# Autodesk Inventor assembly: M2-M-前足
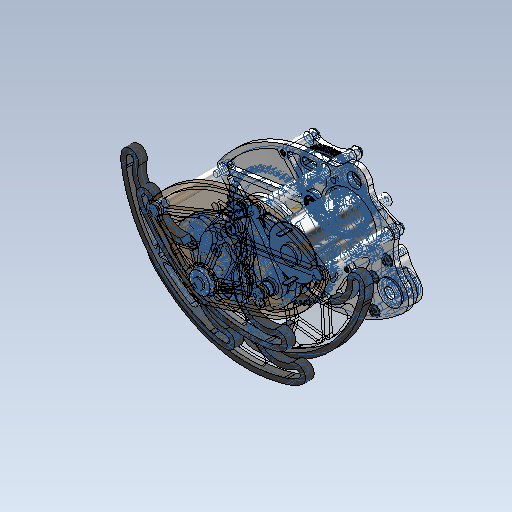
[picture p0: Inventor's stored thumbnail of the model, 512x512]
Saved by Autodesk Inventor 2020 (Build 240168000, 168)
## iProperties
Created: 2021-02-23
Part Number: M2-M-前足
Document SubType Name: Assembly
Designer: AA19065
Mass: 271.583 g
Surface Area: 1202.67 cm^2
Volume: 103.505 cm^3
Density: 2.62385 g/cm^3
Author: AA19065
## Documents named in this file (24)
- C:\Users\happy\OneDrive\ドキュメント\賢一ファイル\SRDC\試作10-2\アセンブリ\M2-M-前足.iam
- C:\Users\happy\OneDrive\ドキュメント\賢一ファイル\SRDC\試作10-2\フレーム\M2-M-前足内側フレームv2.ipt
- C:\Users\happy\OneDrive\ドキュメント\賢一ファイル\SRDC\試作10-2\アセンブリ\M2-M-脚クランク.iam
- C:\Users\happy\OneDrive\ドキュメント\賢一ファイル\SRDC\試作10-2\軸受け\M2-M-オイレスw5f12-14n.ipt
- C:\Users\happy\OneDrive\ドキュメント\賢一ファイル\SRDC\試作10-2\スペーサ\M2-M-40mm.ipt
- C:\Users\happy\OneDrive\ドキュメント\賢一ファイル\SRDC\試作10-2\フレーム\M2-M-前足外側フレームv2.ipt
- C:\Users\happy\OneDrive\ドキュメント\賢一ファイル\SRDC\試作10-2\軸受け\M2-M-φ6φ12ベアリングa.ipt
- C:\Users\happy\OneDrive\ドキュメント\賢一ファイル\SRDC\試作10-2\モータ\M2-M-RS-380.ipt
- C:\Users\happy\OneDrive\ドキュメント\賢一ファイル\SRDC\試作10-2\モータ\M2-M-モータマウントv2.ipt
- C:\Users\happy\OneDrive\ドキュメント\賢一ファイル\SRDC\試作10-2\軸受け\M2-M-φ4φ8ベアリングa.ipt
- C:\Users\happy\OneDrive\ドキュメント\賢一ファイル\SRDC\試作10-2\ピン\M2-M-φ4ピン　L20.ipt
- C:\Users\happy\OneDrive\ドキュメント\賢一ファイル\SRDC\試作10-2\アセンブリ\M2-M-脚ギア1段目.iam
- C:\Users\happy\OneDrive\ドキュメント\賢一ファイル\SRDC\試作10-2\ギア\M2-M-ピニオン10.ipt
- C:\Users\happy\OneDrive\ドキュメント\賢一ファイル\SRDC\試作10-2\ギア\M2-M-m1z60.ipt
- C:\Users\happy\OneDrive\ドキュメント\賢一ファイル\SRDC\試作10-2\ギア\M2-M-脚ギアマウントv3.ipt
- C:\Users\happy\OneDrive\ドキュメント\賢一ファイル\SRDC\試作10-2\脚クランク\原動節v2\M2-M-原動節ギア接続部v2.ipt
- C:\Users\happy\OneDrive\ドキュメント\賢一ファイル\SRDC\試作10-2\ねじ\M2-M-M3ボタンボルト8.ipt
- C:\Users\happy\OneDrive\ドキュメント\賢一ファイル\SRDC\試作10-2\スペーサ\M2-M-12mm.ipt
- C:\Users\happy\OneDrive\ドキュメント\賢一ファイル\SRDC\試作10-2\ねじ\M2-M-M3ボタンボルト18.ipt
- C:\Users\happy\OneDrive\ドキュメント\賢一ファイル\SRDC\試作10-2\ねじ\M2-M-m3皿ネジ12.ipt
- C:\Users\happy\OneDrive\ドキュメント\賢一ファイル\SRDC\試作10-2\フレーム\M2-M-前足フレーム補助パーツ.ipt
- C:\Users\happy\OneDrive\ドキュメント\賢一ファイル\SRDC\試作10-2\ねじ\M2-M-m2.6 6mm キャップボルト.ipt
- C:\Users\happy\OneDrive\ドキュメント\賢一ファイル\SRDC\試作10-2\ねじ\M2-M-M3ボタンボルト20.ipt
- C:\Users\happy\OneDrive\ドキュメント\賢一ファイル\SRDC\試作10-2\スペーサ\M2-18mm.ipt
## Components (45 placed, 23 different names)
1. M2-M-前足内側フレームv2:1 — 挿入:2, 挿入:4, 挿入:3, 挿入:6, 挿入:5, 挿入:12, 挿入:13, 挿入:14, 挿入:37, 挿入:38, 挿入:47, 挿入:43, 挿入:44, 挿入:52, 挿入:53, 挿入:54, 挿入:59, 挿入:58, 挿入:60, 挿入:47
2. M2-M-脚クランク:1 [sub-assembly] — 挿入:1, メイト:1, 挿入:32, 挿入:30, 挿入:31
3. M2-M-オイレスw5f12-14n:1 — 挿入:1, 挿入:2
4. M2-M-40mm:1 — 挿入:4, 挿入:7
5. M2-M-40mm:2 — 挿入:3, メイト:1
6. M2-M-40mm:3 — 挿入:6
7. M2-M-40mm:4 — 挿入:5, 挿入:8
8. M2-M-前足外側フレームv2:1 — 挿入:7, 挿入:8, 挿入:9, 挿入:33, 挿入:34, 挿入:35, 挿入:36
9. M2-M-φ6φ12ベアリングa:1 — 挿入:9
10. M2-M-RS-380:1 — 挿入:10, 挿入:11, 挿入:15
11. M2-M-モータマウントv2:1 — 挿入:10, 挿入:11, 挿入:12, 挿入:13, 挿入:56, 挿入:57, 挿入:61, 挿入:62, 挿入:63
12. M2-M-φ4φ8ベアリングa:1 — 挿入:14, メイト:3, フラッシュ:1, メイト:4
13. M2-M-φ4φ8ベアリングa:2 — メイト:5, 挿入:29
14. M2-M-φ4ピン　L20:1 — メイト:3, フラッシュ:1, メイト:5, メイト:2
15. M2-M-脚ギア1段目:1 [sub-assembly] — メイト:2, メイト:4
16. M2-M-ピニオン10:1 — 挿入:15
17. M2-M-m1z60:1 — 挿入:32, メイト:6
18. M2-M-脚ギアマウントv3:1 — 挿入:29, 挿入:46, 挿入:49, 挿入:50, 挿入:64
19. M2-M-原動節ギア接続部v2:1 — 挿入:30, 挿入:31, メイト:6, 挿入:51
20. M2-M-M3ボタンボルト8:1 — 挿入:33
21. M2-M-M3ボタンボルト8:2 — 挿入:34
22. M2-M-M3ボタンボルト8:3 — 挿入:35
23. M2-M-M3ボタンボルト8:4 — 挿入:36
24. M2-M-M3ボタンボルト8:5 — 挿入:37
25. M2-M-M3ボタンボルト8:6 — 挿入:38
26. M2-M-12mm:1 — 挿入:47
27. M2-M-12mm:2 — 挿入:43, 挿入:46
28. M2-M-12mm:3 — 挿入:44
29. M2-M-M3ボタンボルト18:1 — 挿入:49
30. M2-M-M3ボタンボルト18:2 — 挿入:50
31. M2-M-m3皿ネジ12:1 — 挿入:51
32. M2-M-φ6φ12ベアリングa:2 — 挿入:55
33. M2-M-前足フレーム補助パーツ:1 — 挿入:52, 挿入:53, 挿入:55
34. M2-M-φ6φ12ベアリングa:3 — 挿入:54
35. M2-M-M3ボタンボルト8:7 — 挿入:56
36. M2-M-M3ボタンボルト8:8 — 挿入:57
37. M2-M-M3ボタンボルト8:9
38. M2-M-M3ボタンボルト8:10 — 挿入:59
39. M2-M-M3ボタンボルト8:11 — 挿入:58
40. M2-M-M3ボタンボルト8:12 — 挿入:60
41. M2-M-M3ボタンボルト8:13 — 挿入:61
42. M2-M-m2.6 6mm キャップボルト:1 — 挿入:62
43. M2-M-m2.6 6mm キャップボルト:2 — 挿入:63
44. M2-M-M3ボタンボルト20:1 — 挿入:64
45. M2-18mm:1 — 挿入:47
## Relationships (53: Insert 46, Mate 6, Flush 1)
- 挿入:1 [Insert]: M2-M-脚クランク:1 ↔ M2-M-オイレスw5f12-14n:1
- 挿入:2 [Insert] (0.5 mm): M2-M-前足内側フレームv2:1 ↔ M2-M-オイレスw5f12-14n:1
- 挿入:4 [Insert]: M2-M-前足内側フレームv2:1 ↔ M2-M-40mm:1
- 挿入:3 [Insert]: M2-M-前足内側フレームv2:1 ↔ M2-M-40mm:2
- メイト:1 [Mate]: M2-M-脚クランク:1 ↔ M2-M-40mm:2
- 挿入:6 [Insert]: M2-M-前足内側フレームv2:1 ↔ M2-M-40mm:3
- 挿入:5 [Insert]: M2-M-前足内側フレームv2:1 ↔ M2-M-40mm:4
- 挿入:7 [Insert]: M2-M-40mm:1 ↔ M2-M-前足外側フレームv2:1
- 挿入:8 [Insert]: M2-M-40mm:4 ↔ M2-M-前足外側フレームv2:1
- 挿入:9 [Insert]: M2-M-前足外側フレームv2:1 ↔ M2-M-φ6φ12ベアリングa:1
- 挿入:10 [Insert]: M2-M-RS-380:1 ↔ M2-M-モータマウントv2:1
- 挿入:11 [Insert]: M2-M-RS-380:1 ↔ M2-M-モータマウントv2:1
- 挿入:12 [Insert]: M2-M-前足内側フレームv2:1 ↔ M2-M-モータマウントv2:1
- 挿入:13 [Insert]: M2-M-前足内側フレームv2:1 ↔ M2-M-モータマウントv2:1
- 挿入:14 [Insert]: M2-M-前足内側フレームv2:1 ↔ M2-M-φ4φ8ベアリングa:1
- メイト:3 [Mate]: M2-M-φ4φ8ベアリングa:1 ↔ M2-M-φ4ピン　L20:1
- フラッシュ:1 [Flush]: M2-M-φ4φ8ベアリングa:1 ↔ M2-M-φ4ピン　L20:1
- メイト:5 [Mate]: M2-M-φ4φ8ベアリングa:2 ↔ M2-M-φ4ピン　L20:1
- メイト:2 [Mate]: M2-M-φ4ピン　L20:1 ↔ M2-M-脚ギア1段目:1
- メイト:4 [Mate] (2 mm): M2-M-φ4φ8ベアリングa:1 ↔ M2-M-脚ギア1段目:1
- 挿入:15 [Insert] (1 mm): M2-M-RS-380:1 ↔ M2-M-ピニオン10:1
- 挿入:32 [Insert]: M2-M-脚クランク:1 ↔ M2-M-m1z60:1
- 挿入:29 [Insert]: M2-M-φ4φ8ベアリングa:2 ↔ M2-M-脚ギアマウントv3:1
- 挿入:30 [Insert]: M2-M-脚クランク:1 ↔ M2-M-原動節ギア接続部v2:1
- 挿入:31 [Insert]: M2-M-脚クランク:1 ↔ M2-M-原動節ギア接続部v2:1
- メイト:6 [Mate]: M2-M-m1z60:1 ↔ M2-M-原動節ギア接続部v2:1
- 挿入:33 [Insert]: M2-M-前足外側フレームv2:1 ↔ M2-M-M3ボタンボルト8:1
- 挿入:34 [Insert]: M2-M-前足外側フレームv2:1 ↔ M2-M-M3ボタンボルト8:2
- 挿入:35 [Insert]: M2-M-前足外側フレームv2:1 ↔ M2-M-M3ボタンボルト8:3
- 挿入:36 [Insert]: M2-M-前足外側フレームv2:1 ↔ M2-M-M3ボタンボルト8:4
- 挿入:37 [Insert]: M2-M-前足内側フレームv2:1 ↔ M2-M-M3ボタンボルト8:5
- 挿入:38 [Insert]: M2-M-前足内側フレームv2:1 ↔ M2-M-M3ボタンボルト8:6
- 挿入:47 [Insert]: M2-M-前足内側フレームv2:1 ↔ M2-M-12mm:1
- 挿入:43 [Insert]: M2-M-前足内側フレームv2:1 ↔ M2-M-12mm:2
- 挿入:46 [Insert]: M2-M-脚ギアマウントv3:1 ↔ M2-M-12mm:2
- 挿入:44 [Insert]: M2-M-前足内側フレームv2:1 ↔ M2-M-12mm:3
- 挿入:49 [Insert]: M2-M-脚ギアマウントv3:1 ↔ M2-M-M3ボタンボルト18:1
- 挿入:50 [Insert]: M2-M-脚ギアマウントv3:1 ↔ M2-M-M3ボタンボルト18:2
- 挿入:51 [Insert]: M2-M-原動節ギア接続部v2:1 ↔ M2-M-m3皿ネジ12:1
- 挿入:52 [Insert]: M2-M-前足内側フレームv2:1 ↔ M2-M-前足フレーム補助パーツ:1
- 挿入:53 [Insert]: M2-M-前足内側フレームv2:1 ↔ M2-M-前足フレーム補助パーツ:1
- 挿入:55 [Insert]: M2-M-φ6φ12ベアリングa:2 ↔ M2-M-前足フレーム補助パーツ:1
- 挿入:54 [Insert]: M2-M-前足内側フレームv2:1 ↔ M2-M-φ6φ12ベアリングa:3
- 挿入:56 [Insert]: M2-M-モータマウントv2:1 ↔ M2-M-M3ボタンボルト8:7
- 挿入:57 [Insert]: M2-M-モータマウントv2:1 ↔ M2-M-M3ボタンボルト8:8
- 挿入:59 [Insert]: M2-M-前足内側フレームv2:1 ↔ M2-M-M3ボタンボルト8:10
- 挿入:58 [Insert]: M2-M-前足内側フレームv2:1 ↔ M2-M-M3ボタンボルト8:11
- 挿入:60 [Insert]: M2-M-前足内側フレームv2:1 ↔ M2-M-M3ボタンボルト8:12
- 挿入:61 [Insert]: M2-M-モータマウントv2:1 ↔ M2-M-M3ボタンボルト8:13
- 挿入:62 [Insert]: M2-M-モータマウントv2:1 ↔ M2-M-m2.6 6mm キャップボルト:1
- 挿入:63 [Insert]: M2-M-モータマウントv2:1 ↔ M2-M-m2.6 6mm キャップボルト:2
- 挿入:64 [Insert]: M2-M-脚ギアマウントv3:1 ↔ M2-M-M3ボタンボルト20:1
- 挿入:47 [Insert]: M2-M-前足内側フレームv2:1 ↔ M2-18mm:1
